# Autodesk Inventor assembly: Mid Flaps and Guide Rail Assembly
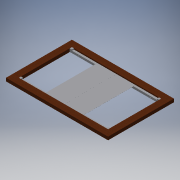
[picture p0: Inventor's stored thumbnail of the model, 180x180]
Saved by Autodesk Inventor 2016 (Build 200138000, 138)
## iProperties
Created: 2016-04-04
Part Number: Mid Flaps and Guide Rail Assembly
Document SubType Name: Assembly
Designer: amycroft3
Author: amycroft3
## Documents named in this file (5)
- C:\Users\Andrea\Documents\Dropbox\Capstone CAD\Mid Flaps and Guide Rail Assembly.iam
- C:\Users\Andrea\Documents\Dropbox\Capstone CAD\Opening flap_Side2Side Motion.ipt
- C:\Users\Andrea\Documents\Dropbox\Capstone CAD\Support GuideRail Wood Framing.ipt
- C:\Users\Andrea\Documents\Dropbox\Capstone CAD\Support GuideRail Wood Framing Joining Piece.ipt
- C:\Users\Andrea\Documents\Dropbox\Capstone CAD\Support GuideRail.ipt
## Components (8 placed, 4 different names)
1. Support GuideRail Wood Framing:1 — Flush:5, Flush:6, Mate:14, Flush:9, Flush:10, Flush:11, Mate:18, Flush:14, Mate:22, Mate:23
2. Support GuideRail Wood Framing:2 — Flush:5, Flush:6, Mate:15, Flush:12, Mate:19
3. Opening flap_Side2Side Motion:1 — Flush:7, Flush:8, Mate:13, Mate:21, Mate:22, Symmetry:1
4. Opening flap_Side2Side Motion:2 — Flush:7, Flush:8, Mate:13, Symmetry:1
5. Support GuideRail Wood Framing Joining Piece:1 — Mate:14, Flush:9, Flush:10, Mate:20
6. Support GuideRail Wood Framing Joining Piece:2 — Mate:15, Flush:11, Flush:12, Mate:23
7. Support GuideRail:1 — Flush:13, Mate:16, Mate:17, Mate:18, Mate:20, Flush:14, Mate:21
8. Support GuideRail:2 — Flush:13, Mate:16, Mate:17, Mate:19
## Relationships (22: Mate 11, Flush 10, Symmetry 1)
- Flush:5: Support GuideRail Wood Framing:1 ↔ Support GuideRail Wood Framing:2
- Flush:6: Support GuideRail Wood Framing:1 ↔ Support GuideRail Wood Framing:2
- Flush:7: Opening flap_Side2Side Motion:1 ↔ Opening flap_Side2Side Motion:2
- Flush:8: Opening flap_Side2Side Motion:1 ↔ Opening flap_Side2Side Motion:2
- Mate:13: Opening flap_Side2Side Motion:1 ↔ Opening flap_Side2Side Motion:2
- Mate:14: Support GuideRail Wood Framing:1 ↔ Support GuideRail Wood Framing Joining Piece:1
- Flush:9: Support GuideRail Wood Framing:1 ↔ Support GuideRail Wood Framing Joining Piece:1
- Flush:10: Support GuideRail Wood Framing:1 ↔ Support GuideRail Wood Framing Joining Piece:1
- Mate:15: Support GuideRail Wood Framing:2 ↔ Support GuideRail Wood Framing Joining Piece:2
- Flush:11: Support GuideRail Wood Framing:1 ↔ Support GuideRail Wood Framing Joining Piece:2
- Flush:12: Support GuideRail Wood Framing:2 ↔ Support GuideRail Wood Framing Joining Piece:2
- Flush:13: Support GuideRail:1 ↔ Support GuideRail:2
- Mate:16: Support GuideRail:1 ↔ Support GuideRail:2
- Mate:17: Support GuideRail:1 ↔ Support GuideRail:2
- Mate:18: Support GuideRail Wood Framing:1 ↔ Support GuideRail:1
- Mate:19: Support GuideRail Wood Framing:2 ↔ Support GuideRail:2
- Mate:20: Support GuideRail Wood Framing Joining Piece:1 ↔ Support GuideRail:1
- Flush:14: Support GuideRail Wood Framing:1 ↔ Support GuideRail:1
- Mate:21: Opening flap_Side2Side Motion:1 ↔ Support GuideRail:1
- Mate:22 (6.35 mm): Support GuideRail Wood Framing:1 ↔ Opening flap_Side2Side Motion:1
- Mate:23: Support GuideRail Wood Framing:1 ↔ Support GuideRail Wood Framing Joining Piece:2
- Symmetry:1: Opening flap_Side2Side Motion:1 ↔ Opening flap_Side2Side Motion:2
